# Autodesk Inventor assembly: X-Gantry Joiner Right V2 Assembly
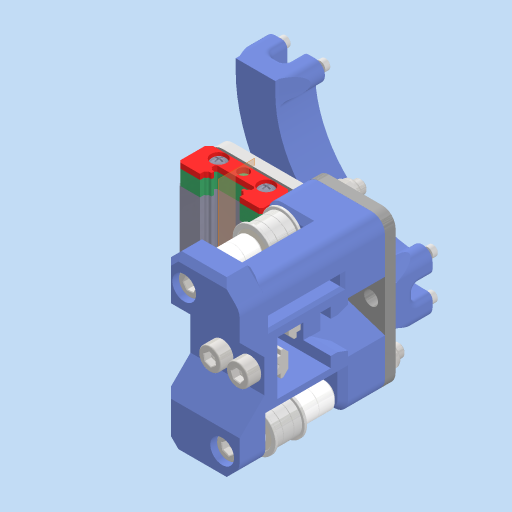
[picture p0: Inventor's stored thumbnail of the model, 512x512]
Saved by Autodesk Inventor 2023.2 (Build 272271000, 271)
## iProperties
Created: 2023-12-06
Part Number: X-Gantry Joiner Right V2 Assembly
Document SubType Name: Assembly
Designer: Nils Bade
Author: Nils Bade
## Documents named in this file (17)
- C:\Users\nilsb\Documents\Inventor\Projektarbeit-Bade\RatRig_Bade\X-Gantry Joiner Right V2 Assembly.iam
- C:\Users\nilsb\Documents\Inventor\Projektarbeit-Bade\RatRig_modified\xy Joiner Right for 4040 V2.ipt
- C:\Users\nilsb\Documents\Inventor\Projektarbeit-Bade\RatRig_modified\XY Joiner Plate for 4040.ipt
- C:\Users\nilsb\Documents\Inventor\Projektarbeit-Bade\RatRig_modified\MGN15 Linear-Rail-Block.ipt
- C:\Users\nilsb\Documents\Inventor\Projektarbeit-Bade\Schrauben\Cap Head Screw M3x12 v2.ipt
- C:\Users\nilsb\Documents\Inventor\Projektarbeit-Bade\RatRig_Standards\T-Nut - Square type for 2020 - M5 v2.ipt
- C:\Users\nilsb\Documents\Inventor\Projektarbeit-Bade\Schrauben\Cap Head Screw M5x10 v2.ipt
- C:\Users\nilsb\Documents\Inventor\Projektarbeit-Bade\Schrauben\Cap Head Screw M5x60.ipt
- C:\Users\nilsb\Documents\Inventor\Projektarbeit-Bade\RatRig_Standards\Hex Locking Nut - M5 v2.ipt
- C:\Users\nilsb\Documents\Inventor\Projektarbeit-Bade\RatRig_Standards\Mini Precision Shim - 8x5x1mm v2.ipt
- C:\Users\nilsb\Documents\Inventor\Projektarbeit-Bade\RatRig_Standards\Ball Bearing - F695ZZ v1.ipt
- C:\Users\nilsb\Documents\Inventor\Projektarbeit-Bade\RatRig_Standards\Ball Bearing - 695ZZ v1.ipt
- C:\Users\nilsb\Documents\Inventor\Projektarbeit-Bade\RatRig_Standards\Aluminium Spacer - 6mm v2.ipt
- C:\Users\nilsb\Documents\Inventor\Projektarbeit-Bade\RatRig_modified\HF-Kabelführung X-Gantry Base.ipt
- C:\Users\nilsb\Documents\Inventor\Projektarbeit-Bade\Schrauben\Cap Head Screw M4x8 - DIN912.ipt
- C:\Users\nilsb\Documents\Inventor\Projektarbeit-Bade\RatRig_modified\HF-Kabelführung X-Gantry Deckel.ipt
- C:\Users\nilsb\Documents\Inventor\Projektarbeit-Bade\Schrauben\Cap Head Screw M2x6 - DIN912.ipt
## Components (41 placed, 16 different names)
1. xy Joiner Right for 4040 V2:1 — Passend:49, Passend:50, Passend:51, Passend:63, Passend:65, Passend:66, Passend:67, Passend:68, Passend:70, Passend:71, Passend:72, Passend:74, Passend:75, Passend:76, Passend:79, Passend:80, Passend:81, Passend:82
2. XY Joiner Plate for 4040:1 — Passend:49, Passend:50, Passend:51, Passend:52, Passend:53, Passend:54, Passend:55, Passend:56, Passend:57, Passend:58, Passend:59, Passend:60, Passend:61, Passend:62, Passend:64, Passend:69, Passend:83, Passend:85, Passend:86, Passend:87
3. MGN15 Linear-Rail-Block:1 — Passend:52, Passend:53, Passend:54
4. Cap Head Screw M3x12 v2:1 — Passend:56, Passend:61
5. Cap Head Screw M3x12 v2:2 — Passend:55, Passend:62
6. Cap Head Screw M3x12 v2:3 — Passend:58, Passend:59
7. Cap Head Screw M3x12 v2:4 — Passend:57, Passend:60
8. T-Nut - Square type for 2020 - M5 v2:1 — Passend:73, Passend:74
9. T-Nut - Square type for 2020 - M5 v2:2 — Passend:78, Passend:80
10. T-Nut - Square type for 2020 - M5 v2:3 — Passend:77, Passend:79
11. Cap Head Screw M5x10 v2:1 — Passend:75, Passend:78, Passend:82
12. Cap Head Screw M5x10 v2:2 — Passend:76, Passend:77, Passend:81
13. Cap Head Screw M5x60:1 — Passend:63, Passend:66
14. Cap Head Screw M5x60:2 — Passend:67, Passend:70
15. Hex Locking Nut - M5 v2:1 — Passend:64
16. Hex Locking Nut - M5 v2:2 — Passend:69
17. Mini Precision Shim - 8x5x1mm v2:1
18. Mini Precision Shim - 8x5x1mm v2:2
19. Mini Precision Shim - 8x5x1mm v2:3 — Passend:68
20. Mini Precision Shim - 8x5x1mm v2:4
21. Mini Precision Shim - 8x5x1mm v2:5
22. Mini Precision Shim - 8x5x1mm v2:6 — Passend:65
23. Ball Bearing - F695ZZ v1:1
24. Ball Bearing - F695ZZ v1:2
25. Ball Bearing - F695ZZ v1:3
26. Ball Bearing - F695ZZ v1:4
27. Ball Bearing - 695ZZ v1:1
28. Ball Bearing - 695ZZ v1:2
29. Aluminium Spacer - 6mm v2:1
30. Aluminium Spacer - 6mm v2:2
31. Aluminium Spacer - 6mm v2:3
32. Aluminium Spacer - 6mm v2:4
33. Cap Head Screw M5x10 v2:3 — Passend:71, Passend:72, Passend:73
34. HF-Kabelführung X-Gantry Base:1 — Passend:85, Passend:86, Passend:87, Passend:88, Passend:91, Passend:92, Passend:93, Passend:94, Passend:95
35. Cap Head Screw M4x8 - DIN912:1 — Passend:88, Passend:91
36. Cap Head Screw M4x8 - DIN912:2 — Passend:83, Passend:95
37. HF-Kabelführung X-Gantry Deckel:1 — Passend:92, Passend:93, Passend:94, Passend:96, Passend:97, Passend:98, Passend:99, Passend:100, Passend:101, Passend:102, Passend:103
38. Cap Head Screw M2x6 - DIN912:1 — Passend:96, Passend:100
39. Cap Head Screw M2x6 - DIN912:2 — Passend:97, Passend:101
40. Cap Head Screw M2x6 - DIN912:3 — Passend:98, Passend:103
41. Cap Head Screw M2x6 - DIN912:4 — Passend:99, Passend:102
## Relationships (86: Mate 86)
- [Mate]: Cap Head Screw M5x60:1 ↔ Hex Locking Nut - M5 v2:1
- [Mate]: Cap Head Screw M5x60:2 ↔ Hex Locking Nut - M5 v2:2
- [Mate]: Cap Head Screw M5x60:2 ↔ Mini Precision Shim - 8x5x1mm v2:3
- [Mate]: Cap Head Screw M5x60:2 ↔ Ball Bearing - F695ZZ v1:4
- [Mate]: Mini Precision Shim - 8x5x1mm v2:3 ↔ Ball Bearing - F695ZZ v1:4
- [Mate]: Cap Head Screw M5x60:2 ↔ Ball Bearing - 695ZZ v1:1
- [Mate]: Ball Bearing - F695ZZ v1:4 ↔ Ball Bearing - 695ZZ v1:1
- [Mate]: Cap Head Screw M5x60:2 ↔ Ball Bearing - F695ZZ v1:1
- [Mate]: Ball Bearing - F695ZZ v1:1 ↔ Ball Bearing - 695ZZ v1:1
- [Mate]: Cap Head Screw M5x60:2 ↔ Mini Precision Shim - 8x5x1mm v2:2
- [Mate]: Mini Precision Shim - 8x5x1mm v2:2 ↔ Ball Bearing - F695ZZ v1:1
- [Mate]: Cap Head Screw M5x60:2 ↔ Aluminium Spacer - 6mm v2:1
- [Mate]: Mini Precision Shim - 8x5x1mm v2:2 ↔ Aluminium Spacer - 6mm v2:1
- [Mate]: Cap Head Screw M5x60:2 ↔ Aluminium Spacer - 6mm v2:2
- [Mate]: Aluminium Spacer - 6mm v2:1 ↔ Aluminium Spacer - 6mm v2:2
- [Mate]: Cap Head Screw M5x60:2 ↔ Mini Precision Shim - 8x5x1mm v2:1
- [Mate]: Mini Precision Shim - 8x5x1mm v2:1 ↔ Aluminium Spacer - 6mm v2:2
- [Mate]: Cap Head Screw M5x60:1 ↔ Mini Precision Shim - 8x5x1mm v2:4
- [Mate]: Cap Head Screw M5x60:1 ↔ Ball Bearing - F695ZZ v1:2
- [Mate]: Mini Precision Shim - 8x5x1mm v2:4 ↔ Ball Bearing - F695ZZ v1:2
- [Mate]: Cap Head Screw M5x60:1 ↔ Ball Bearing - 695ZZ v1:2
- [Mate]: Ball Bearing - F695ZZ v1:2 ↔ Ball Bearing - 695ZZ v1:2
- [Mate]: Cap Head Screw M5x60:1 ↔ Ball Bearing - F695ZZ v1:3
- [Mate]: Ball Bearing - F695ZZ v1:3 ↔ Ball Bearing - 695ZZ v1:2
- [Mate]: Cap Head Screw M5x60:1 ↔ Mini Precision Shim - 8x5x1mm v2:5
- [Mate]: Mini Precision Shim - 8x5x1mm v2:5 ↔ Ball Bearing - F695ZZ v1:3
- [Mate]: Cap Head Screw M5x60:1 ↔ Aluminium Spacer - 6mm v2:3
- [Mate]: Mini Precision Shim - 8x5x1mm v2:5 ↔ Aluminium Spacer - 6mm v2:3
- [Mate]: Cap Head Screw M5x60:1 ↔ Aluminium Spacer - 6mm v2:4
- [Mate]: Aluminium Spacer - 6mm v2:3 ↔ Aluminium Spacer - 6mm v2:4
- [Mate]: Cap Head Screw M5x60:1 ↔ Mini Precision Shim - 8x5x1mm v2:6
- [Mate]: Mini Precision Shim - 8x5x1mm v2:6 ↔ Aluminium Spacer - 6mm v2:4
- [Mate]: T-Nut - Square type for 2020 - M5 v2:2 ↔ Cap Head Screw M5x10 v2:1
- [Mate]: T-Nut - Square type for 2020 - M5 v2:3 ↔ Cap Head Screw M5x10 v2:2
- Passend:49 [Mate]: xy Joiner Right for 4040 V2:1 ↔ XY Joiner Plate for 4040:1
- Passend:50 [Mate]: xy Joiner Right for 4040 V2:1 ↔ XY Joiner Plate for 4040:1
- Passend:51 [Mate]: xy Joiner Right for 4040 V2:1 ↔ XY Joiner Plate for 4040:1
- Passend:52 [Mate]: XY Joiner Plate for 4040:1 ↔ MGN15 Linear-Rail-Block:1
- Passend:53 [Mate]: XY Joiner Plate for 4040:1 ↔ MGN15 Linear-Rail-Block:1
- Passend:54 [Mate]: XY Joiner Plate for 4040:1 ↔ MGN15 Linear-Rail-Block:1
- Passend:55 [Mate]: XY Joiner Plate for 4040:1 ↔ Cap Head Screw M3x12 v2:2
- Passend:56 [Mate]: XY Joiner Plate for 4040:1 ↔ Cap Head Screw M3x12 v2:1
- Passend:57 [Mate]: XY Joiner Plate for 4040:1 ↔ Cap Head Screw M3x12 v2:4
- Passend:58 [Mate]: XY Joiner Plate for 4040:1 ↔ Cap Head Screw M3x12 v2:3
- Passend:59 [Mate]: XY Joiner Plate for 4040:1 ↔ Cap Head Screw M3x12 v2:3
- Passend:60 [Mate]: XY Joiner Plate for 4040:1 ↔ Cap Head Screw M3x12 v2:4
- Passend:61 [Mate]: XY Joiner Plate for 4040:1 ↔ Cap Head Screw M3x12 v2:1
- Passend:62 [Mate]: XY Joiner Plate for 4040:1 ↔ Cap Head Screw M3x12 v2:2
- Passend:63 [Mate]: xy Joiner Right for 4040 V2:1 ↔ Cap Head Screw M5x60:1
- Passend:64 [Mate]: XY Joiner Plate for 4040:1 ↔ Hex Locking Nut - M5 v2:1
- Passend:65 [Mate]: xy Joiner Right for 4040 V2:1 ↔ Mini Precision Shim - 8x5x1mm v2:6
- Passend:66 [Mate]: xy Joiner Right for 4040 V2:1 ↔ Cap Head Screw M5x60:1
- Passend:67 [Mate]: xy Joiner Right for 4040 V2:1 ↔ Cap Head Screw M5x60:2
- Passend:68 [Mate]: xy Joiner Right for 4040 V2:1 ↔ Mini Precision Shim - 8x5x1mm v2:3
- Passend:69 [Mate]: XY Joiner Plate for 4040:1 ↔ Hex Locking Nut - M5 v2:2
- Passend:70 [Mate]: xy Joiner Right for 4040 V2:1 ↔ Cap Head Screw M5x60:2
- Passend:71 [Mate]: xy Joiner Right for 4040 V2:1 ↔ Cap Head Screw M5x10 v2:3
- Passend:72 [Mate]: xy Joiner Right for 4040 V2:1 ↔ Cap Head Screw M5x10 v2:3
- Passend:73 [Mate]: T-Nut - Square type for 2020 - M5 v2:1 ↔ Cap Head Screw M5x10 v2:3
- Passend:74 [Mate] (1.8 mm): xy Joiner Right for 4040 V2:1 ↔ T-Nut - Square type for 2020 - M5 v2:1
- Passend:75 [Mate]: xy Joiner Right for 4040 V2:1 ↔ Cap Head Screw M5x10 v2:1
- Passend:76 [Mate]: xy Joiner Right for 4040 V2:1 ↔ Cap Head Screw M5x10 v2:2
- Passend:77 [Mate]: T-Nut - Square type for 2020 - M5 v2:3 ↔ Cap Head Screw M5x10 v2:2
- Passend:78 [Mate]: T-Nut - Square type for 2020 - M5 v2:2 ↔ Cap Head Screw M5x10 v2:1
- Passend:79 [Mate] (1.8 mm): xy Joiner Right for 4040 V2:1 ↔ T-Nut - Square type for 2020 - M5 v2:3
- Passend:80 [Mate] (1.8 mm): xy Joiner Right for 4040 V2:1 ↔ T-Nut - Square type for 2020 - M5 v2:2
- Passend:81 [Mate]: xy Joiner Right for 4040 V2:1 ↔ Cap Head Screw M5x10 v2:2
- Passend:82 [Mate]: xy Joiner Right for 4040 V2:1 ↔ Cap Head Screw M5x10 v2:1
- Passend:83 [Mate]: XY Joiner Plate for 4040:1 ↔ Cap Head Screw M4x8 - DIN912:2
- Passend:85 [Mate]: XY Joiner Plate for 4040:1 ↔ HF-Kabelführung X-Gantry Base:1
- Passend:86 [Mate]: XY Joiner Plate for 4040:1 ↔ HF-Kabelführung X-Gantry Base:1
- Passend:87 [Mate]: XY Joiner Plate for 4040:1 ↔ HF-Kabelführung X-Gantry Base:1
- Passend:88 [Mate]: HF-Kabelführung X-Gantry Base:1 ↔ Cap Head Screw M4x8 - DIN912:1
- Passend:91 [Mate]: HF-Kabelführung X-Gantry Base:1 ↔ Cap Head Screw M4x8 - DIN912:1
- Passend:92 [Mate]: HF-Kabelführung X-Gantry Base:1 ↔ HF-Kabelführung X-Gantry Deckel:1
- Passend:93 [Mate]: HF-Kabelführung X-Gantry Base:1 ↔ HF-Kabelführung X-Gantry Deckel:1
- Passend:94 [Mate]: HF-Kabelführung X-Gantry Base:1 ↔ HF-Kabelführung X-Gantry Deckel:1
- Passend:95 [Mate]: HF-Kabelführung X-Gantry Base:1 ↔ Cap Head Screw M4x8 - DIN912:2
- Passend:96 [Mate]: HF-Kabelführung X-Gantry Deckel:1 ↔ Cap Head Screw M2x6 - DIN912:1
- Passend:97 [Mate]: HF-Kabelführung X-Gantry Deckel:1 ↔ Cap Head Screw M2x6 - DIN912:2
- Passend:98 [Mate]: HF-Kabelführung X-Gantry Deckel:1 ↔ Cap Head Screw M2x6 - DIN912:3
- Passend:99 [Mate]: HF-Kabelführung X-Gantry Deckel:1 ↔ Cap Head Screw M2x6 - DIN912:4
- Passend:100 [Mate]: HF-Kabelführung X-Gantry Deckel:1 ↔ Cap Head Screw M2x6 - DIN912:1
- Passend:101 [Mate]: HF-Kabelführung X-Gantry Deckel:1 ↔ Cap Head Screw M2x6 - DIN912:2
- Passend:102 [Mate]: HF-Kabelführung X-Gantry Deckel:1 ↔ Cap Head Screw M2x6 - DIN912:4
- Passend:103 [Mate]: HF-Kabelführung X-Gantry Deckel:1 ↔ Cap Head Screw M2x6 - DIN912:3
## Named parameters: d25_d36 = 0 mm, d5_d37 = 0 mm, d8_d40 = 0 mm, d9_d42 = 0 mm, d10_d43 = 0 mm, d11_d44 = 0 mm
